# Autodesk Inventor assembly: Mark 6 - Final Preseason
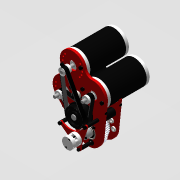
[picture p0: Inventor's stored thumbnail of the model, 180x180]
Saved by Autodesk Inventor 2013 (Build 170138000, 138)
## iProperties
Created: 2013-08-20
Part Number: Mark 6 - Final Preseason
Document SubType Name: Assembly
Designer: grtstudent
Author: grtstudent
## Documents named in this file (50)
- C:\Users\grtstudent\Desktop\Mark 6 Final Preseason\Mark 6 - Final Preseason.iam
- C:\Users\grtstudent\Desktop\Mark 5\Bearings\R10-2RS.ipt
- C:\Users\grtstudent\Desktop\Mark 6 Final Preseason\Bearings\R10-Open.ipt
- C:\Users\grtstudent\Desktop\Mark 6 Final Preseason\Shafts\Output Shaft\Output Shaft Bushing.ipt
- C:\Users\grtstudent\Desktop\Mark 6 Final Preseason\Shafts\Output Shaft\Output Shaft.ipt
- C:\Users\grtstudent\Desktop\Mark 6 Final Preseason\Shafts\Output Shaft\35T 20DP - .188 Ball Shifting Bore.ipt
- C:\Users\grtstudent\Desktop\Mark 6 Final Preseason\Shafts\Output Shaft\48T 20DP - .188 Ball Shifting Bore.ipt
- C:\Users\grtstudent\Desktop\Mark 6 Final Preseason\Bearings\Thrust Bearing Washer - .6250 Bore.ipt
- C:\Users\grtstudent\Desktop\Mark 6 Final Preseason\Plates\Cim Plate\Cim Plate.ipt
- C:\Users\grtstudent\Desktop\Mark 6 Final Preseason\Plates\Mounting Plate\Main Connecting Standoff Thick.ipt
- C:\Users\grtstudent\Desktop\Mark 6 Final Preseason\Plates\Pneumatic Plate\Pnuematic Plate.ipt
- C:\Users\grtstudent\Desktop\Mark 6 Final Preseason\Motors\Rotor.ipt
- C:\Users\grtstudent\Desktop\Mark 6 Final Preseason\Motors\CIM Can.ipt
- C:\Users\grtstudent\Desktop\Mark 6 Final Preseason\Motors\Mini CIM Can.ipt
- C:\Users\grtstudent\Desktop\Mark 6 Final Preseason\Bearings\FR6-2RS.ipt
- C:\Users\grtstudent\Desktop\Mark 6 Final Preseason\Bearings\FR8-2RS.ipt
- C:\Users\grtstudent\Desktop\Mark 6 Final Preseason\Shafts\Cluster Shaft\Cluster Shaft.ipt
- C:\Users\grtstudent\Desktop\Mark 6 Final Preseason\Shafts\Cluster Shaft\15T 20DP - .375 Hex Bore.ipt
- C:\Users\grtstudent\Desktop\Mark 6 Final Preseason\Shafts\Cluster Shaft\28T 20DP - .375 Hex Bore.ipt
- C:\Users\grtstudent\Desktop\Mark 6 Final Preseason\Shafts\Cluster Shaft\Cluster Shaft Spacer.ipt
- C:\Users\grtstudent\Desktop\Mark 6 Final Preseason\Pulleys\16T 3mm GT2 - 8mm Key Broach.ipt
- C:\Users\grtstudent\Desktop\Mark 6 Final Preseason\Belts\285 mm Belt.ipt
- C:\Users\grtstudent\Desktop\Final Preseason\Belts\267mm Belt.ipt
- C:\Users\grtstudent\Desktop\Mark 6 Final Preseason\Pneumatic\Pancake Pneumatic.iam
- C:\Users\grtstudent\Desktop\Mark 6 Final Preseason\Bearings\R4-2RS.ipt
- C:\Users\grtstudent\Desktop\Mark 6 Final Preseason\Plates\Pneumatic Plate\4-40 Clinch Style Pem Nut .091 Minimum Panel Thickness.ipt
- C:\Users\grtstudent\Desktop\Mark 6 Final Preseason\Bolts\Button Head Cap Screw 8-32 Thread .250 Length.ipt
- C:\Users\grtstudent\Desktop\Mark 6 Final Preseason\Encoder\S4-120-250-N-S-B.ipt
- C:\Users\grtstudent\Desktop\Mark 6 Final Preseason\Bearings\R3-2RS.ipt
- C:\Users\grtstudent\Desktop\Mark 6 Final Preseason\Pneumatic\Pneumatic Connector.ipt
- C:\Users\grtstudent\Desktop\Mark 6 Final Preseason\Pneumatic\Pneumatic Connector Cap.ipt
- C:\Users\grtstudent\Desktop\Final Preseason\Bolts\Button Head Cap Screw 4-40 Thread .500 Length.ipt
- C:\Users\grtstudent\Desktop\Mark 6 Final Preseason\Plates\Pneumatic Plate\Supporting Plate Standoff Thin.ipt
- C:\Users\grtstudent\Desktop\Mark 6 Final Preseason\Plates\Pneumatic Plate\Supporting Plate Standoff Thick.ipt
- C:\Users\grtstudent\Desktop\Final Preseason\Shafts\Ball Shifting Shaft.ipt
- C:\Users\grtstudent\Desktop\Final Preseason\Spring Pin 1-16 Diameter.ipt
- C:\Users\grtstudent\Desktop\Mark 6 Final Preseason\Bolts\Socket Head Cap Screw 4-40 Thread 1.125 Length.ipt
- C:\Users\grtstudent\Desktop\Mark 6 Final Preseason\Shafts\Cluster Shaft\48T 3mm GT2 Plastic - .500 Hex Broach.ipt
- C:\Users\grtstudent\Desktop\Mark 6 Final Preseason\Bolts\Socket Head Cap Screw 10-32 Thread 3.000 Length.ipt
- C:\Users\grtstudent\Desktop\Mark 6 Final Preseason\Plates\Mounting Plate\Main Connecting Standoff Stepped.ipt
- C:\Users\grtstudent\Desktop\Mark 6 Final Preseason\Plates\Mounting Plate\Mounting Plate Mark 7.ipt
- C:\Users\grtstudent\Desktop\Mark 6 Final Preseason\Plates\Mounting Plate\10-32 Flush Mounted Pem Nut.ipt
- C:\Users\grtstudent\Desktop\Mark 6 Final Preseason\Bolts\Socket Head Cap Screw 10-32 Thread 2.500 Length.ipt
- C:\Users\grtstudent\Desktop\Mark 6 Final Preseason\Bolts\Socket Head Cap Screw 10-32 Thread .500 Length.ipt
- C:\Users\grtstudent\Desktop\Mark 6 Final Preseason\Bolts\Socket Head Cap Screw 8-32 Thread 1.500 Length.ipt
- C:\Users\grtstudent\Desktop\Mark 6 Final Preseason\Encoder\Encoder Mount.ipt
- C:\Users\grtstudent\Desktop\Mark 6 Final Preseason\Bolts\Socket Head Cap Screw 6-32 Thread .500 Length.ipt
- C:\Users\grtstudent\Desktop\Mark 6 Final Preseason\Bolts\Socket Head Cap Screw 8-32 Thread .375 Length.ipt
- C:\Users\grtstudent\Desktop\Mark 6 Final Preseason\Bolts\Button Head Cap Screw 6-32 Thread .250 Length.ipt
- C:\Users\grtstudent\Desktop\Mark 6 Final Preseason\Plates\Mounting Plate\.25-20 Pem Nut.ipt
## Components (80 placed, 49 different names)
1. Mounting Plate Mark 7:1 — Mate:212, Flush:6, Mate:213, Mate:214, Mate:216, Mate:217, Mate:219, Mate:220, Mate:225, Mate:226, Mate:227, Mate:228, Mate:229, Mate:230, Mate:242, Mate:243, Mate:244, Mate:254, Mate:262, Mate:263, Mate:264, Mate:265, Mate:274, Mate:275, Mate:276, Mate:277, Mate:280, Mate:282
2. R10-2RS:1 — Mate:18, Mate:24
3. R10-Open:1 — Mate:6, Mate:7, Mate:9
4. R10-2RS:2 — Mate:2, Mate:3, Flush:6, Mate:213
5. R10-Open:2 — Mate:12, Mate:15, Mate:21
6. Output Shaft Bushing:1 — Mate:4, Mate:5
7. Output Shaft:1 — Mate:2, Mate:3, Mate:4, Mate:5, Mate:6, Mate:7, Mate:8, Mate:12, Mate:14, Mate:18, Mate:19, Mate:22, Flush:7
8. 35T 20DP - .188 Ball Shifting Bore:1 — Mate:8, Mate:9, Mate:20, Flush:3
9. 48T 20DP - .188 Ball Shifting Bore:1 — Mate:14, Mate:15, Mate:23
10. Thrust Bearing Washer - .6250 Bore:1 — Mate:19, Mate:20, Mate:21
11. Thrust Bearing Washer - .6250 Bore:2 — Mate:22, Mate:23, Mate:24
12. Cim Plate:1 — Mate:158, Mate:159, Mate:160, Mate:161, Mate:169, Mate:178, Mate:185, Mate:188, Mate:189, Mate:190, Mate:192, Mate:205, Mate:206, Mate:207, Mate:208, Mate:209, Mate:210, Flush:7, Mate:231, Mate:234, Mate:235, Mate:236, Mate:237, Mate:238, Mate:239, Mate:255, Mate:278, Mate:281
13. Main Connecting Standoff Thick:1 — Mate:160, Mate:161, Mate:212
14. Main Connecting Standoff Thick:2 — Mate:158, Mate:159
15. Main Connecting Standoff Stepped:1 — Mate:209, Mate:210, Mate:211, Mate:232, Mate:233
16. Pnuematic Plate:1 — Mate:105, Mate:106, Mate:107, Mate:114, Mate:115, Mate:116, Mate:117, Mate:135, Mate:136, Mate:139, Mate:191, Mate:193, Mate:194, Mate:196, Mate:197, Mate:240, Mate:241, Mate:283, Mate:284
17. Rotor:1 — Mate:47, Mate:49, Mate:81, Mate:90
18. Rotor:2 — Mate:83, Mate:89, Mate:170, Mate:171
19. Rotor:3 — Mate:82, Mate:88, Mate:186, Mate:187
20. CIM Can:1 — Mate:47, Mate:49, Mate:178
21. CIM Can:2 — Mate:185, Mate:186, Mate:187
22. Mini CIM Can:1 — Mate:169, Mate:170, Mate:171
23. FR6-2RS:1 — Mate:72, Mate:215, Mate:216
24. FR8-2RS:1 — Mate:54, Mate:55, Mate:58, Mate:154, Mate:188
25. Cluster Shaft:1 — Mate:54, Mate:55, Mate:57, Mate:60, Mate:70, Mate:71, Mate:73, Mate:86, Mate:91, Mate:122, Mate:123, Mate:152, Mate:153, Mate:155, Mate:156, Mate:214, Mate:215
26. 15T 20DP - .375 Hex Bore:1 — Mate:57, Mate:58, Mate:70
27. 28T 20DP - .375 Hex Bore:1 — Mate:60, Mate:71, Flush:3
28. Cluster Shaft Spacer:1 — Mate:72, Mate:73
29. 16T 3mm GT2 - 8mm Key Broach:1 — Mate:81, Flush:5
30. 16T 3mm GT2 - 8mm Key Broach:2 — Mate:83, Flush:4
31. 16T 3mm GT2 - 8mm Key Broach:3 — Mate:82, Mate:204
32. 285 mm Belt:1 — Mate:86, Mate:88, Mate:200, Mate:204
33. 267mm Belt:1 — Mate:89, Mate:90, Mate:91, Mate:201, Flush:4, Flush:5
34. Socket Head Cap Screw 10-32 Thread .500 Length:1 — Mate:239
35. Socket Head Cap Screw 10-32 Thread .500 Length:2 — Mate:236
36. Socket Head Cap Screw 10-32 Thread .500 Length:3 — Mate:238
37. Socket Head Cap Screw 10-32 Thread .500 Length:4 — Mate:234
38. Socket Head Cap Screw 10-32 Thread .500 Length:5 — Mate:237
39. Socket Head Cap Screw 10-32 Thread .500 Length:6 — Mate:235
40. Pancake Pneumatic:1 [sub-assembly] — Mate:105, Mate:106, Mate:107, Mate:124, Mate:125, Mate:127, Mate:148, Mate:149, Mate:150, Mate:151
41. R4-2RS:1 — Mate:110, Mate:111, Mate:202
42. R4-2RS:2 — Mate:110, Mate:111, Mate:211
43. 4-40 Clinch Style Pem Nut .091 Minimum Panel Thickness:1 — Mate:114, Mate:115
44. 4-40 Clinch Style Pem Nut .091 Minimum Panel Thickness:2 — Mate:116, Mate:117
45. Button Head Cap Screw 8-32 Thread .250 Length:1 — Mate:205, Mate:207
46. Button Head Cap Screw 8-32 Thread .250 Length:2 — Mate:206, Mate:208
47. S4-120-250-N-S-B:1 — Mate:122, Mate:123
48. R3-2RS:1 — Mate:124, Mate:126, Mate:147
49. Pneumatic Connector:1 — Mate:125, Mate:126, Mate:127, Mate:128, Mate:129, Mate:130, Mate:131, Mate:132, Mate:133, Mate:134, Mate:249, Mate:250
50. Pneumatic Connector Cap:1 — Mate:128, Mate:129, Mate:130, Mate:142
51. Button Head Cap Screw 4-40 Thread .500 Length:1 — Mate:133, Mate:134, Mate:284
52. Button Head Cap Screw 4-40 Thread .500 Length:2 — Mate:131, Mate:132, Mate:283
53. Supporting Plate Standoff Thin:1 — Mate:136, Mate:139, Mate:192, Mate:195
54. Supporting Plate Standoff Thin:2 — Mate:135, Mate:189, Mate:190, Mate:191
55. Supporting Plate Standoff Thick:1 — Mate:193, Mate:231
56. Ball Shifting Shaft:1 — Mate:142, Mate:145, Mate:146, Mate:147
57. Spring Pin 1-16 Diameter:1 — Mate:145, Mate:146
58. Socket Head Cap Screw 4-40 Thread 1.125 Length:1 — Mate:148, Mate:150
59. Socket Head Cap Screw 4-40 Thread 1.125 Length:2 — Mate:149, Mate:151
60. 48T 3mm GT2 Plastic - .500 Hex Broach:1 — Mate:155, Mate:156, Mate:157, Mate:200
61. 48T 3mm GT2 Plastic - .500 Hex Broach:2 — Mate:152, Mate:153, Mate:154, Mate:157, Mate:201, Mate:202
62. Socket Head Cap Screw 10-32 Thread 3.000 Length:1 — Mate:195, Mate:197
63. Socket Head Cap Screw 10-32 Thread 3.000 Length:2 — Mate:194, Mate:196
64. 10-32 Flush Mounted Pem Nut:1 — Mate:220, Mate:229, Mate:230
65. 10-32 Flush Mounted Pem Nut:2 — Mate:217, Mate:227, Mate:228
66. 10-32 Flush Mounted Pem Nut:3 — Mate:219, Mate:225, Mate:226
67. Socket Head Cap Screw 10-32 Thread 2.500 Length:1 — Mate:232, Mate:233
68. Socket Head Cap Screw 8-32 Thread 1.500 Length:1 — Mate:240, Mate:241
69. Encoder Mount:1 — Mate:242, Mate:243, Mate:244, Mate:245, Mate:246, Mate:247, Mate:248
70. Socket Head Cap Screw 6-32 Thread .500 Length:1 — Mate:245, Mate:248
71. Socket Head Cap Screw 6-32 Thread .500 Length:2 — Mate:246, Mate:247
72. Socket Head Cap Screw 8-32 Thread .375 Length:1 — Mate:249, Mate:250
73. Button Head Cap Screw 6-32 Thread .250 Length:1 — Mate:278, Mate:281
74. Button Head Cap Screw 6-32 Thread .250 Length:2 — Mate:280, Mate:282
75. Button Head Cap Screw 6-32 Thread .250 Length:3 — Mate:254
76. Button Head Cap Screw 6-32 Thread .250 Length:4 — Mate:255
77. .25-20 Pem Nut:1 — Mate:264, Mate:274
78. .25-20 Pem Nut:2 — Mate:263, Mate:276
79. .25-20 Pem Nut:3 — Mate:262, Mate:277
80. .25-20 Pem Nut:4 — Mate:265, Mate:275
## Relationships (175: Mate 170, Flush 5)
- Mate:2: R10-2RS:2 ↔ Output Shaft:1
- Mate:3: R10-2RS:2 ↔ Output Shaft:1
- Mate:4: Output Shaft Bushing:1 ↔ Output Shaft:1
- Mate:5: Output Shaft Bushing:1 ↔ Output Shaft:1
- Mate:6: R10-Open:1 ↔ Output Shaft:1
- Mate:7: R10-Open:1 ↔ Output Shaft:1
- Mate:8: Output Shaft:1 ↔ 35T 20DP - .188 Ball Shifting Bore:1
- Mate:9: R10-Open:1 ↔ 35T 20DP - .188 Ball Shifting Bore:1
- Mate:12: R10-Open:2 ↔ Output Shaft:1
- Mate:14: Output Shaft:1 ↔ 48T 20DP - .188 Ball Shifting Bore:1
- Mate:15: R10-Open:2 ↔ 48T 20DP - .188 Ball Shifting Bore:1
- Mate:18: R10-2RS:1 ↔ Output Shaft:1
- Mate:19: Output Shaft:1 ↔ Thrust Bearing Washer - .6250 Bore:1
- Mate:20: 35T 20DP - .188 Ball Shifting Bore:1 ↔ Thrust Bearing Washer - .6250 Bore:1
- Mate:21: R10-Open:2 ↔ Thrust Bearing Washer - .6250 Bore:1
- Mate:22: Output Shaft:1 ↔ Thrust Bearing Washer - .6250 Bore:2
- Mate:23: 48T 20DP - .188 Ball Shifting Bore:1 ↔ Thrust Bearing Washer - .6250 Bore:2
- Mate:24: R10-2RS:1 ↔ Thrust Bearing Washer - .6250 Bore:2
- Mate:47: Rotor:1 ↔ CIM Can:1
- Mate:49: Rotor:1 ↔ CIM Can:1
- Mate:54: FR8-2RS:1 ↔ Cluster Shaft:1
- Mate:55: FR8-2RS:1 ↔ Cluster Shaft:1
- Mate:57: Cluster Shaft:1 ↔ 15T 20DP - .375 Hex Bore:1
- Mate:58: FR8-2RS:1 ↔ 15T 20DP - .375 Hex Bore:1
- Mate:60: Cluster Shaft:1 ↔ 28T 20DP - .375 Hex Bore:1
- Mate:70: Cluster Shaft:1 ↔ 15T 20DP - .375 Hex Bore:1
- Mate:71: Cluster Shaft:1 ↔ 28T 20DP - .375 Hex Bore:1
- Flush:3: 35T 20DP - .188 Ball Shifting Bore:1 ↔ 28T 20DP - .375 Hex Bore:1
- Mate:72: FR6-2RS:1 ↔ Cluster Shaft Spacer:1
- Mate:73: Cluster Shaft:1 ↔ Cluster Shaft Spacer:1
- Mate:81: Rotor:1 ↔ 16T 3mm GT2 - 8mm Key Broach:1
- Mate:82: Rotor:3 ↔ 16T 3mm GT2 - 8mm Key Broach:3
- Mate:83: Rotor:2 ↔ 16T 3mm GT2 - 8mm Key Broach:2
- Mate:86: Cluster Shaft:1 ↔ 285 mm Belt:1
- Mate:88: Rotor:3 ↔ 285 mm Belt:1
- Mate:89: Rotor:2 ↔ 267mm Belt:1
- Mate:90: Rotor:1 ↔ 267mm Belt:1
- Mate:91: Cluster Shaft:1 ↔ 267mm Belt:1
- Mate:105: Pnuematic Plate:1 ↔ Pancake Pneumatic:1
- Mate:106: Pnuematic Plate:1 ↔ Pancake Pneumatic:1
- Mate:107: Pnuematic Plate:1 ↔ Pancake Pneumatic:1
- Mate:110: R4-2RS:1 ↔ R4-2RS:2
- Mate:111: R4-2RS:1 ↔ R4-2RS:2
- Mate:114: Pnuematic Plate:1 ↔ 4-40 Clinch Style Pem Nut .091 Minimum Panel Thickness:1
- Mate:115: Pnuematic Plate:1 ↔ 4-40 Clinch Style Pem Nut .091 Minimum Panel Thickness:1
- Mate:116: Pnuematic Plate:1 ↔ 4-40 Clinch Style Pem Nut .091 Minimum Panel Thickness:2
- Mate:117: Pnuematic Plate:1 ↔ 4-40 Clinch Style Pem Nut .091 Minimum Panel Thickness:2
- Mate:122: Cluster Shaft:1 ↔ S4-120-250-N-S-B:1
- Mate:123 (0.254 mm): Cluster Shaft:1 ↔ S4-120-250-N-S-B:1
- Mate:124: Pancake Pneumatic:1 ↔ R3-2RS:1
- Mate:125: Pancake Pneumatic:1 ↔ Pneumatic Connector:1
- Mate:126: R3-2RS:1 ↔ Pneumatic Connector:1
- Mate:127: Pancake Pneumatic:1 ↔ Pneumatic Connector:1
- Mate:128: Pneumatic Connector:1 ↔ Pneumatic Connector Cap:1
- Mate:129: Pneumatic Connector:1 ↔ Pneumatic Connector Cap:1
- Mate:130: Pneumatic Connector:1 ↔ Pneumatic Connector Cap:1
- Mate:131: Pneumatic Connector:1 ↔ Button Head Cap Screw 4-40 Thread .500 Length:2
- Mate:132: Pneumatic Connector:1 ↔ Button Head Cap Screw 4-40 Thread .500 Length:2
- Mate:133: Pneumatic Connector:1 ↔ Button Head Cap Screw 4-40 Thread .500 Length:1
- Mate:134: Pneumatic Connector:1 ↔ Button Head Cap Screw 4-40 Thread .500 Length:1
- Mate:135: Pnuematic Plate:1 ↔ Supporting Plate Standoff Thin:2
- Mate:136: Pnuematic Plate:1 ↔ Supporting Plate Standoff Thin:1
- Mate:139: Pnuematic Plate:1 ↔ Supporting Plate Standoff Thin:1
- Mate:142: Pneumatic Connector Cap:1 ↔ Ball Shifting Shaft:1
- Mate:145: Ball Shifting Shaft:1 ↔ Spring Pin 1-16 Diameter:1
- Mate:146: Ball Shifting Shaft:1 ↔ Spring Pin 1-16 Diameter:1
- Mate:147: R3-2RS:1 ↔ Ball Shifting Shaft:1
- Mate:148: Pancake Pneumatic:1 ↔ Socket Head Cap Screw 4-40 Thread 1.125 Length:1
- Mate:149: Pancake Pneumatic:1 ↔ Socket Head Cap Screw 4-40 Thread 1.125 Length:2
- Mate:150: Pancake Pneumatic:1 ↔ Socket Head Cap Screw 4-40 Thread 1.125 Length:1
- Mate:151: Pancake Pneumatic:1 ↔ Socket Head Cap Screw 4-40 Thread 1.125 Length:2
- Mate:152: Cluster Shaft:1 ↔ 48T 3mm GT2 Plastic - .500 Hex Broach:2
- Mate:153: Cluster Shaft:1 ↔ 48T 3mm GT2 Plastic - .500 Hex Broach:2
- Mate:154: FR8-2RS:1 ↔ 48T 3mm GT2 Plastic - .500 Hex Broach:2
- Mate:155: Cluster Shaft:1 ↔ 48T 3mm GT2 Plastic - .500 Hex Broach:1
- Mate:156: Cluster Shaft:1 ↔ 48T 3mm GT2 Plastic - .500 Hex Broach:1
- Mate:157: 48T 3mm GT2 Plastic - .500 Hex Broach:1 ↔ 48T 3mm GT2 Plastic - .500 Hex Broach:2
- Mate:158: Cim Plate:1 ↔ Main Connecting Standoff Thick:2
- Mate:159: Cim Plate:1 ↔ Main Connecting Standoff Thick:2
- Mate:160: Cim Plate:1 ↔ Main Connecting Standoff Thick:1
- Mate:161: Cim Plate:1 ↔ Main Connecting Standoff Thick:1
- [Mate]: Cim Plate:1 ↔ Socket Head Cap Screw 10-32 Thread .500 Length:1
- [Mate]: Cim Plate:1 ↔ Socket Head Cap Screw 10-32 Thread .500 Length:3
- [Mate]: Mini CIM Can:1 ↔ Socket Head Cap Screw 10-32 Thread .500 Length:1
- [Mate]: Mini CIM Can:1 ↔ Socket Head Cap Screw 10-32 Thread .500 Length:3
- Mate:169: Cim Plate:1 ↔ Mini CIM Can:1
- Mate:170: Rotor:2 ↔ Mini CIM Can:1
- Mate:171: Rotor:2 ↔ Mini CIM Can:1
- [Mate]: Cim Plate:1 ↔ Socket Head Cap Screw 10-32 Thread .500 Length:6
- [Mate]: Cim Plate:1 ↔ Socket Head Cap Screw 10-32 Thread .500 Length:4
- [Mate]: CIM Can:1 ↔ Socket Head Cap Screw 10-32 Thread .500 Length:4
- [Mate]: CIM Can:1 ↔ Socket Head Cap Screw 10-32 Thread .500 Length:6
- Mate:178: Cim Plate:1 ↔ CIM Can:1
- [Mate]: Cim Plate:1 ↔ Socket Head Cap Screw 10-32 Thread .500 Length:2
- [Mate]: Cim Plate:1 ↔ Socket Head Cap Screw 10-32 Thread .500 Length:5
- [Mate]: CIM Can:2 ↔ Socket Head Cap Screw 10-32 Thread .500 Length:2
- [Mate]: CIM Can:2 ↔ Socket Head Cap Screw 10-32 Thread .500 Length:5
- Mate:185: Cim Plate:1 ↔ CIM Can:2
- Mate:186: Rotor:3 ↔ CIM Can:2
- Mate:187: Rotor:3 ↔ CIM Can:2
- Mate:188: Cim Plate:1 ↔ FR8-2RS:1
- Mate:189: Cim Plate:1 ↔ Supporting Plate Standoff Thin:2
- Mate:190: Cim Plate:1 ↔ Supporting Plate Standoff Thin:2
- Mate:191: Pnuematic Plate:1 ↔ Supporting Plate Standoff Thin:2
- Mate:192: Cim Plate:1 ↔ Supporting Plate Standoff Thin:1
- Mate:193: Pnuematic Plate:1 ↔ Supporting Plate Standoff Thick:1
- Mate:194: Pnuematic Plate:1 ↔ Socket Head Cap Screw 10-32 Thread 3.000 Length:2
- Mate:195: Supporting Plate Standoff Thin:1 ↔ Socket Head Cap Screw 10-32 Thread 3.000 Length:1
- Mate:196: Pnuematic Plate:1 ↔ Socket Head Cap Screw 10-32 Thread 3.000 Length:2
- Mate:197: Pnuematic Plate:1 ↔ Socket Head Cap Screw 10-32 Thread 3.000 Length:1
- Mate:200: 285 mm Belt:1 ↔ 48T 3mm GT2 Plastic - .500 Hex Broach:1
- Mate:201: 267mm Belt:1 ↔ 48T 3mm GT2 Plastic - .500 Hex Broach:2
- Mate:202: R4-2RS:1 ↔ 48T 3mm GT2 Plastic - .500 Hex Broach:2
- Mate:204: 16T 3mm GT2 - 8mm Key Broach:3 ↔ 285 mm Belt:1
- Flush:4: 16T 3mm GT2 - 8mm Key Broach:2 ↔ 267mm Belt:1
- Flush:5: 16T 3mm GT2 - 8mm Key Broach:1 ↔ 267mm Belt:1
- Mate:205: Cim Plate:1 ↔ Button Head Cap Screw 8-32 Thread .250 Length:1
- Mate:206: Cim Plate:1 ↔ Button Head Cap Screw 8-32 Thread .250 Length:2
- Mate:207: Cim Plate:1 ↔ Button Head Cap Screw 8-32 Thread .250 Length:1
- Mate:208: Cim Plate:1 ↔ Button Head Cap Screw 8-32 Thread .250 Length:2
- Mate:209: Cim Plate:1 ↔ Main Connecting Standoff Stepped:1
- Mate:210: Cim Plate:1 ↔ Main Connecting Standoff Stepped:1
- Mate:211: Main Connecting Standoff Stepped:1 ↔ R4-2RS:2
- Mate:212: Mounting Plate Mark 7:1 ↔ Main Connecting Standoff Thick:1
- Flush:6: Mounting Plate Mark 7:1 ↔ R10-2RS:2
- Mate:213: Mounting Plate Mark 7:1 ↔ R10-2RS:2
- Mate:214: Mounting Plate Mark 7:1 ↔ Cluster Shaft:1
- Flush:7: Output Shaft:1 ↔ Cim Plate:1
- Mate:215: FR6-2RS:1 ↔ Cluster Shaft:1
- Mate:216: Mounting Plate Mark 7:1 ↔ FR6-2RS:1
- Mate:217: Mounting Plate Mark 7:1 ↔ 10-32 Flush Mounted Pem Nut:2
- Mate:219: Mounting Plate Mark 7:1 ↔ 10-32 Flush Mounted Pem Nut:3
- Mate:220: Mounting Plate Mark 7:1 ↔ 10-32 Flush Mounted Pem Nut:1
- Mate:225: Mounting Plate Mark 7:1 ↔ 10-32 Flush Mounted Pem Nut:3
- Mate:226: Mounting Plate Mark 7:1 ↔ 10-32 Flush Mounted Pem Nut:3
- Mate:227: Mounting Plate Mark 7:1 ↔ 10-32 Flush Mounted Pem Nut:2
- Mate:228: Mounting Plate Mark 7:1 ↔ 10-32 Flush Mounted Pem Nut:2
- Mate:229: Mounting Plate Mark 7:1 ↔ 10-32 Flush Mounted Pem Nut:1
- Mate:230: Mounting Plate Mark 7:1 ↔ 10-32 Flush Mounted Pem Nut:1
- Mate:231: Cim Plate:1 ↔ Supporting Plate Standoff Thick:1
- Mate:232: Main Connecting Standoff Stepped:1 ↔ Socket Head Cap Screw 10-32 Thread 2.500 Length:1
- Mate:233: Main Connecting Standoff Stepped:1 ↔ Socket Head Cap Screw 10-32 Thread 2.500 Length:1
- Mate:234: Cim Plate:1 ↔ Socket Head Cap Screw 10-32 Thread .500 Length:4
- Mate:235: Cim Plate:1 ↔ Socket Head Cap Screw 10-32 Thread .500 Length:6
- Mate:236: Cim Plate:1 ↔ Socket Head Cap Screw 10-32 Thread .500 Length:2
- Mate:237: Cim Plate:1 ↔ Socket Head Cap Screw 10-32 Thread .500 Length:5
- Mate:238: Cim Plate:1 ↔ Socket Head Cap Screw 10-32 Thread .500 Length:3
- Mate:239: Cim Plate:1 ↔ Socket Head Cap Screw 10-32 Thread .500 Length:1
- Mate:240: Pnuematic Plate:1 ↔ Socket Head Cap Screw 8-32 Thread 1.500 Length:1
- Mate:241: Pnuematic Plate:1 ↔ Socket Head Cap Screw 8-32 Thread 1.500 Length:1
- Mate:242: Mounting Plate Mark 7:1 ↔ Encoder Mount:1
- Mate:243: Mounting Plate Mark 7:1 ↔ Encoder Mount:1
- Mate:244: Mounting Plate Mark 7:1 ↔ Encoder Mount:1
- Mate:245: Encoder Mount:1 ↔ Socket Head Cap Screw 6-32 Thread .500 Length:1
- Mate:246: Encoder Mount:1 ↔ Socket Head Cap Screw 6-32 Thread .500 Length:2
- Mate:247: Encoder Mount:1 ↔ Socket Head Cap Screw 6-32 Thread .500 Length:2
- Mate:248: Encoder Mount:1 ↔ Socket Head Cap Screw 6-32 Thread .500 Length:1
- Mate:249: Pneumatic Connector:1 ↔ Socket Head Cap Screw 8-32 Thread .375 Length:1
- Mate:250: Pneumatic Connector:1 ↔ Socket Head Cap Screw 8-32 Thread .375 Length:1
- Mate:254: Mounting Plate Mark 7:1 ↔ Button Head Cap Screw 6-32 Thread .250 Length:3
- Mate:255: Cim Plate:1 ↔ Button Head Cap Screw 6-32 Thread .250 Length:4
- Mate:262: Mounting Plate Mark 7:1 ↔ .25-20 Pem Nut:3
- Mate:263: Mounting Plate Mark 7:1 ↔ .25-20 Pem Nut:2
- Mate:264: Mounting Plate Mark 7:1 ↔ .25-20 Pem Nut:1
- Mate:265: Mounting Plate Mark 7:1 ↔ .25-20 Pem Nut:4
- Mate:274: Mounting Plate Mark 7:1 ↔ .25-20 Pem Nut:1
- Mate:275: Mounting Plate Mark 7:1 ↔ .25-20 Pem Nut:4
- Mate:276: Mounting Plate Mark 7:1 ↔ .25-20 Pem Nut:2
- Mate:277: Mounting Plate Mark 7:1 ↔ .25-20 Pem Nut:3
- Mate:278: Cim Plate:1 ↔ Button Head Cap Screw 6-32 Thread .250 Length:1
- Mate:280: Mounting Plate Mark 7:1 ↔ Button Head Cap Screw 6-32 Thread .250 Length:2
- Mate:281 (0.7937 mm): Cim Plate:1 ↔ Button Head Cap Screw 6-32 Thread .250 Length:1
- Mate:282 (0.7937 mm): Mounting Plate Mark 7:1 ↔ Button Head Cap Screw 6-32 Thread .250 Length:2
- Mate:283: Pnuematic Plate:1 ↔ Button Head Cap Screw 4-40 Thread .500 Length:2
- Mate:284: Pnuematic Plate:1 ↔ Button Head Cap Screw 4-40 Thread .500 Length:1
